# Autodesk Inventor assembly: Bumper assembly
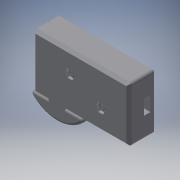
[picture p0: Inventor's stored thumbnail of the model, 180x180]
Saved by Autodesk Inventor 2019 (Build 230136000, 136)
## iProperties
Created: 2018-12-04
Part Number: Bumper assembly
Document SubType Name: Assembly
Designer: Varga Daniel
Author: Varga Daniel
## Documents named in this file (7)
- C:\!_Dani\!_cloud\OneDrive\!_munka\Revolution\RevvyDemoKit\Structural parts\Demo parts\Bumper\Bumper assembly.iam
- C:\!_Dani\!_cloud\OneDrive\!_munka\Revolution\RevvyDemoKit\Structural parts\Demo parts\Bumper\Microswitch\MicroSwitch_internal v2.iam
- C:\!_Dani\!_cloud\OneDrive\!_dokumentumok\Inventor\Content Center Files\R2019\en-US\DIN 7985 (H)\DIN 7985 (H) - M3x16-H.ipt
- C:\!_Dani\!_cloud\OneDrive\!_dokumentumok\Inventor\Content Center Files\R2019\en-US\DIN EN ISO 4032\DIN EN ISO 4032 - M3.ipt
- C:\!_Dani\!_cloud\OneDrive\!_munka\Revolution\RevvyDemoKit\Structural parts\Demo parts\Bumper\bumper cover lower.ipt
- C:\!_Dani\!_cloud\OneDrive\!_munka\Revolution\RevvyDemoKit\Structural parts\Demo parts\Bumper\bumper cover upper.ipt
- C:\!_Dani\!_cloud\OneDrive\!_munka\Revolution\RevvyDemoKit\Structural parts\Demo parts\Bumper\bumper rod.ipt
## Components (8 placed, 6 different names)
1. MicroSwitch_internal v2:1 [sub-assembly] — Mate:1, Mate:2, Mate:5, Flush:4, Flush:5
2. DIN 7985 (H) M3x16-H:1 — Mate:2, Mate:4, Flush:2, Flush:3
3. DIN 7985 (H) M3x16-H:2 — Mate:1, Mate:3, Flush:1, Flush:3, Mate:5
4. DIN EN ISO 4032 M3:1 — Mate:4, Flush:2
5. DIN EN ISO 4032 M3:2 — Mate:3, Flush:1
6. bumper cover lower:1 — Flush:4
7. bumper cover upper:1 — Flush:5, Flush:6
8. bumper rod:1 — Flush:6
## Relationships (11: Flush 6, Mate 5)
- Mate:1: MicroSwitch_internal v2:1 ↔ DIN 7985 (H) M3x16-H:2
- Mate:2: MicroSwitch_internal v2:1 ↔ DIN 7985 (H) M3x16-H:1
- Mate:3: DIN 7985 (H) M3x16-H:2 ↔ DIN EN ISO 4032 M3:2
- Flush:1: DIN 7985 (H) M3x16-H:2 ↔ DIN EN ISO 4032 M3:2
- Mate:4: DIN 7985 (H) M3x16-H:1 ↔ DIN EN ISO 4032 M3:1
- Flush:2: DIN 7985 (H) M3x16-H:1 ↔ DIN EN ISO 4032 M3:1
- Flush:3: DIN 7985 (H) M3x16-H:1 ↔ DIN 7985 (H) M3x16-H:2
- Mate:5 (1.7 mm): MicroSwitch_internal v2:1 ↔ DIN 7985 (H) M3x16-H:2
- Flush:4: MicroSwitch_internal v2:1 ↔ bumper cover lower:1
- Flush:5: MicroSwitch_internal v2:1 ↔ bumper cover upper:1
- Flush:6: bumper cover upper:1 ↔ bumper rod:1
